# Autodesk Inventor assembly: Leg_Loadpipe_Mount
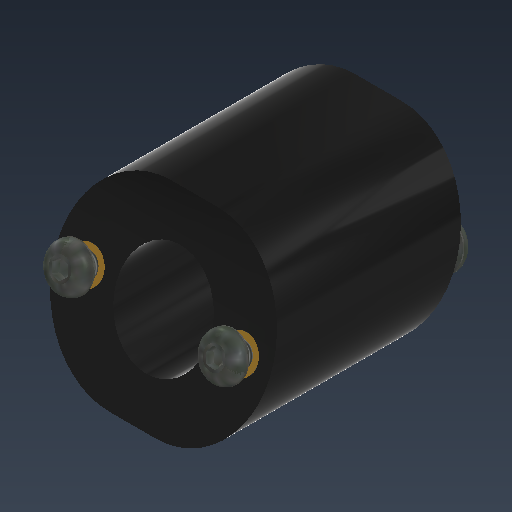
[picture p0: Inventor's stored thumbnail of the model, 512x512]
Saved by Autodesk Inventor 2024.1 (Build 281209000, 209)
## iProperties
Created: 2023-12-05
Part Number: Leg_Loadpipe_Mount
Document SubType Name: Assembly
Designer: dzw04
Mass: 13.5119 g
Surface Area: 52.362 cm^2
Volume: 9.36662 cm^3
Density: 1.44255 g/cm^3
Author: dzw04
## Documents named in this file (6)
- C:\Users\dzw04\Saxion\Mechatronica Lectoraat LMECH LED - Database ARG\Component_Database\SARAX\01. CAD\01. 3D_Drawing\02. Sub_Assemblies\Landing_Gear\02. Sub_Assemblies\Leg_Loadpipe_Mount.iam
- C:\Users\dzw04\Saxion\Mechatronica Lectoraat LMECH LED - Database ARG\Component_Database\SARAX\01. CAD\01. 3D_Drawing\02. Sub_Assemblies\Landing_Gear\01. Parts\Leg_Loadpipe_Mount.ipt
- C:\Users\dzw04\Saxion\Mechatronica Lectoraat LMECH LED - Database ARG\Component_Database\SARAX\01. CAD\01. 3D_Drawing\01. Parts\Threaded_Insert_M3x4.ipt
- C:\Users\dzw04\Saxion\Mechatronica Lectoraat LMECH LED - Database ARG\Component_Database\SARAX\01. CAD\01. 3D_Drawing\01. Parts\en-US\ISO 4026\ISO 4026 - M3 x 4 - ISO.ipt
- C:\Users\dzw04\Saxion\Mechatronica Lectoraat LMECH LED - Database ARG\Component_Database\SARAX\01. CAD\01. 3D_Drawing\01. Parts\en-US\ISO 7380-1\ISO 7380-1 - M3 x 6.ipt
- C:\Users\dzw04\Saxion\Mechatronica Lectoraat LMECH LED - Database ARG\Component_Database\SARAX\01. CAD\01. 3D_Drawing\Parameters.xlsx
## Components (11 placed, 4 different names)
1. Leg_Loadpipe_Mount:1 — Flush:1, Mate:1, Flush:2, Mate:2, Flush:3, Mate:3, Flush:4, Mate:4, Flush:5, Mate:5, Mate:7, Mate:8, Mate:9, Mate:10
2. Threaded_Insert_M3x4:1 — Flush:1, Mate:1, Mate:12
3. Threaded_Insert_M3x4:2 — Flush:2, Mate:2, Mate:11
4. Threaded_Insert_M3x4:3 — Flush:5, Mate:5, Mate:6, Flush:6
5. Threaded_Insert_M3x4:4 — Flush:4, Mate:4, Mate:13
6. Threaded_Insert_M3x4:5 — Flush:3, Mate:3, Mate:14
7. ISO 4026 M3 x 4:1 — Mate:6, Flush:6
8. ISO 7380-1 M3 x 6:1 — Mate:7, Mate:14
9. ISO 7380-1 M3 x 6:2 — Mate:8, Mate:13
10. ISO 7380-1 M3 x 6:3 — Mate:10, Mate:11
11. ISO 7380-1 M3 x 6:4 — Mate:9, Mate:12
## Relationships (20: Mate 14, Flush 6)
- Flush:1: Leg_Loadpipe_Mount:1 ↔ Threaded_Insert_M3x4:1
- Mate:1: Leg_Loadpipe_Mount:1 ↔ Threaded_Insert_M3x4:1
- Flush:2: Leg_Loadpipe_Mount:1 ↔ Threaded_Insert_M3x4:2
- Mate:2: Leg_Loadpipe_Mount:1 ↔ Threaded_Insert_M3x4:2
- Flush:3: Leg_Loadpipe_Mount:1 ↔ Threaded_Insert_M3x4:5
- Mate:3: Leg_Loadpipe_Mount:1 ↔ Threaded_Insert_M3x4:5
- Flush:4: Leg_Loadpipe_Mount:1 ↔ Threaded_Insert_M3x4:4
- Mate:4: Leg_Loadpipe_Mount:1 ↔ Threaded_Insert_M3x4:4
- Flush:5: Leg_Loadpipe_Mount:1 ↔ Threaded_Insert_M3x4:3
- Mate:5: Leg_Loadpipe_Mount:1 ↔ Threaded_Insert_M3x4:3
- Mate:6: Threaded_Insert_M3x4:3 ↔ ISO 4026 M3 x 4:1
- Mate:7 (2.1 mm): Leg_Loadpipe_Mount:1 ↔ ISO 7380-1 M3 x 6:1
- Mate:8 (2.1 mm): Leg_Loadpipe_Mount:1 ↔ ISO 7380-1 M3 x 6:2
- Mate:9 (2 mm): Leg_Loadpipe_Mount:1 ↔ ISO 7380-1 M3 x 6:4
- Mate:10 (2 mm): Leg_Loadpipe_Mount:1 ↔ ISO 7380-1 M3 x 6:3
- Mate:11: Threaded_Insert_M3x4:2 ↔ ISO 7380-1 M3 x 6:3
- Mate:12: Threaded_Insert_M3x4:1 ↔ ISO 7380-1 M3 x 6:4
- Mate:13: Threaded_Insert_M3x4:4 ↔ ISO 7380-1 M3 x 6:2
- Mate:14: Threaded_Insert_M3x4:5 ↔ ISO 7380-1 M3 x 6:1
- Flush:6: Threaded_Insert_M3x4:3 ↔ ISO 4026 M3 x 4:1
## Named parameters: NumberOfArms = 4, RotorToRotor = 900 mm, MountToMotorCenter = 0 mm, ArmPosition = 5 deg, LoadpipeLength = 450 mm, NumberOfBatterys = 2, BatteryLength = 200 mm, BatteryWidth = 62 mm, BatteryHeight = 76 mm, ThicknessBodyOuterPlate = 2 mm, ThicknessBodyCenterPlate = 2 mm, ThicknessLegLoadpipePlate = 2 mm, ThicknessBatteryTray = 2 mm, ThicknessBatteryTopTray = 1 mm, LandingGearHeight = 400 mm, LandingGearStabilityBar = 525 mm, LandingGearRod = 390 mm, StartAngleArm = 45 deg, MotorMountCenter = 71.5 mm
